# Autodesk Inventor assembly: xRailVertcialExtension1inchGap
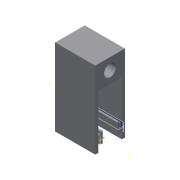
[picture p0: Inventor's stored thumbnail of the model, 180x180]
Saved by Autodesk Inventor 2018 (Build 220112000, 112)
## iProperties
Created: 2019-02-14
Part Number: xRailVertcialExtension1inchGap
Document SubType Name: Assembly
Designer: ball
Author: ball
## Documents named in this file (4)
- C:\FTC\FTC8863CAD\2018Robot\xRailVertcialExtension1inchGap.iam
- C:\FTC\FTC8863CAD\Actobotics\565 parts\565034.ipt
- C:\FTC\FTC8863CAD\Actobotics\585 parts\585757_filled_in.ipt
- C:\FTC\FTC8863CAD\2018Robot\XRailVerticalExtension.ipt
## Components (4 placed, 3 different names)
1. 585757_filled_in:1 — Mate:3, Mate:4, Flush:3, Flush:5
2. 585757_filled_in:2 — Mate:1, Flush:2, Mate:2, Flush:4
3. 565034:1 — Mate:1, Flush:2, Mate:2, Mate:3, Mate:4, Flush:3
4. XRailVerticalExtension:1 — Flush:4, Flush:5
## Relationships (8: Mate 4, Flush 4)
- Mate:1: 585757_filled_in:2 ↔ 565034:1
- Flush:2: 585757_filled_in:2 ↔ 565034:1
- Mate:2: 585757_filled_in:2 ↔ 565034:1
- Mate:3: 585757_filled_in:1 ↔ 565034:1
- Mate:4: 585757_filled_in:1 ↔ 565034:1
- Flush:3: 585757_filled_in:1 ↔ 565034:1
- Flush:4: 585757_filled_in:2 ↔ XRailVerticalExtension:1
- Flush:5: 585757_filled_in:1 ↔ XRailVerticalExtension:1
